# Autodesk Inventor assembly: FrameV2
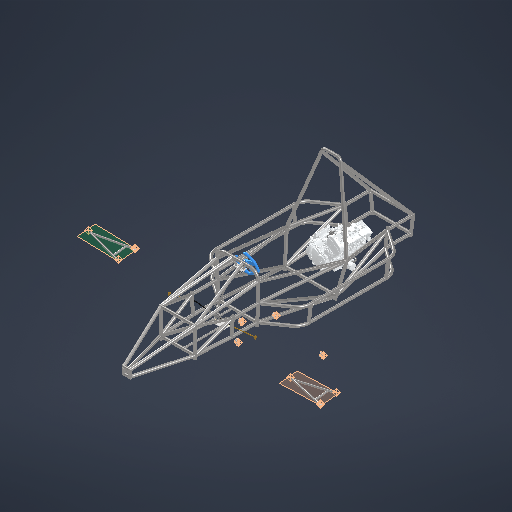
[picture p0: Inventor's stored thumbnail of the model, 512x512]
Saved by Autodesk Inventor 2026.1 (Build 301233000, 233)
## iProperties
Created: 2026-06-05
Part Number: FrameV2
Document SubType Name: Assembly
Designer: tasle
_SolveAssemblyDoc: Frame Generator Solve Assembly
_Version: 15.0.0
Author: tasle
## Documents named in this file (11)
- C:\Users\share\OneDrive\Documents\Personal Projects\GOGO Kart\CAD\GOGO_KART_FSAE\FrameV2.iam
- C:\Users\share\OneDrive\Documents\Personal Projects\GOGO Kart\CAD\GOGO_KART_FSAE\PrelimFrame.ipt
- C:\Users\share\OneDrive\Documents\Personal Projects\GOGO Kart\CAD\GOGO_KART_FSAE\FrameV2\Frame\Frame 1780692296746.iam
- C:\Users\share\OneDrive\Documents\Personal Projects\GOGO Kart\CAD\GOGO_KART_FSAE\honda-cbr600-f4i-engine-1.snapshot.3\Honda CBR600 F4i\Honda CBR600 F4i\Honda CBR600 F4i.ipt
- C:\Users\share\OneDrive\Documents\Personal Projects\GOGO Kart\CAD\GOGO_KART_FSAE\Suspension\Suspension Parts\Front Upper Arm\Front_Upper_Arm_Assembly.iam
- C:\Users\share\OneDrive\Documents\Personal Projects\GOGO Kart\CAD\GOGO_KART_FSAE\Steering\SteeringAssy.iam
- C:\Users\share\OneDrive\Documents\Personal Projects\GOGO Kart\CAD\GOGO_KART_FSAE\Steering\steeringmountplate.ipt
- C:\Users\share\OneDrive\Documents\Personal Projects\GOGO Kart\CAD\GOGO_KART_FSAE\Steering\steeringbracket.ipt
- C:\Users\share\OneDrive\Documents\Personal Projects\GOGO Kart\CAD\GOGO_KART_FSAE\Steering\rackmountplate.ipt
- C:\Users\share\OneDrive\Documents\Personal Projects\GOGO Kart\CAD\GOGO_KART_FSAE\Steering\rackbracket.ipt
- C:\Users\share\OneDrive\Documents\Personal Projects\GOGO Kart\CAD\GOGO_KART_FSAE\Suspension\ALLSTAR 0.5 in Rod End Bracket (Rough).ipt
## Components (15 placed, 10 different names)
1. PrelimFrame:1 — Rotational:3
2. Frame 1780692296746:1 [sub-assembly]
3. Honda CBR600 F4i:1
4. Front_Upper_Arm_Assembly:2 [sub-assembly]
5. SteeringAssy:1 [sub-assembly] — Rigid:1
6. steeringmountplate:1 — Rotational:3, Mate:1, Mate:2, Mate:3
7. steeringbracket:1 — Mate:1, Mate:2, Mate:3, Rigid:1
8. rackmountplate:1 — Rigid:2, Rigid:3
9. rackbracket:1 — Rigid:3
10. rackbracket:2 — Rigid:2
11. ALLSTAR 0.5 in Rod End Bracket (Rough):1
12. ALLSTAR 0.5 in Rod End Bracket (Rough):3
13. ALLSTAR 0.5 in Rod End Bracket (Rough):4
14. ALLSTAR 0.5 in Rod End Bracket (Rough):5
15. Front_Upper_Arm_Assembly:3 [sub-assembly]
## Relationships (7: Mate 3, WeldJoint 3, RevoluteJoint 1)
- Rotational:3 [RevoluteJoint] (-20 mm): PrelimFrame:1 ↔ steeringmountplate:1
- Mate:1: steeringmountplate:1 ↔ steeringbracket:1
- Mate:2: steeringmountplate:1 ↔ steeringbracket:1
- Mate:3: steeringmountplate:1 ↔ steeringbracket:1
- Rigid:1 [WeldJoint]: SteeringAssy:1 ↔ steeringbracket:1
- Rigid:2 [WeldJoint]: rackmountplate:1 ↔ rackbracket:2
- Rigid:3 [WeldJoint]: rackmountplate:1 ↔ rackbracket:1
